# Autodesk Inventor assembly: Assieme1
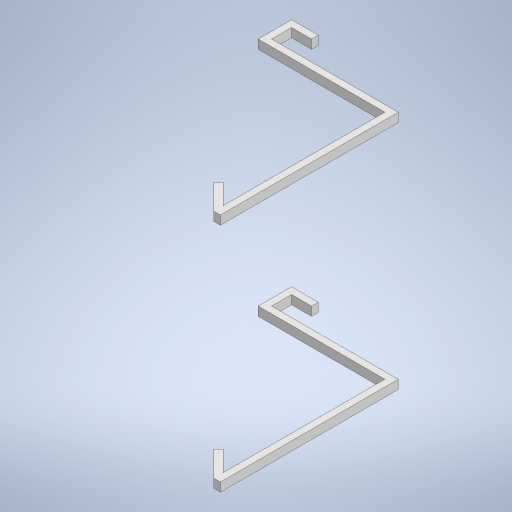
[picture p0: Inventor's stored thumbnail of the model, 512x512]
Saved by Autodesk Inventor 2024 (Build 280153000, 153)
## iProperties
Created: 2024-01-04
Part Number: Assieme1
Document SubType Name: Assembly
Designer: Leonardo
Author: Leonardo
## Documents named in this file (2)
- C:\Users\Leonardo\Documents\Monopattino\Assieme1.iam
- C:\Users\Leonardo\Documents\Monopattino\Staffa.ipt
## Components (2 placed, 1 different names)
1. Staffa:1 — Allineato:3, Allineato:4, Coincidente:4
2. Staffa:2 — Allineato:3, Allineato:4, Coincidente:4
## Relationships (3: Flush 2, Mate 1)
- Allineato:3 [Flush]: Staffa:1 ↔ Staffa:2
- Allineato:4 [Flush]: Staffa:1 ↔ Staffa:2
- Coincidente:4 [Mate] (500 mm): Staffa:1 ↔ Staffa:2
